# Autodesk Inventor assembly: ASY GBK 1310 long wall shield 4
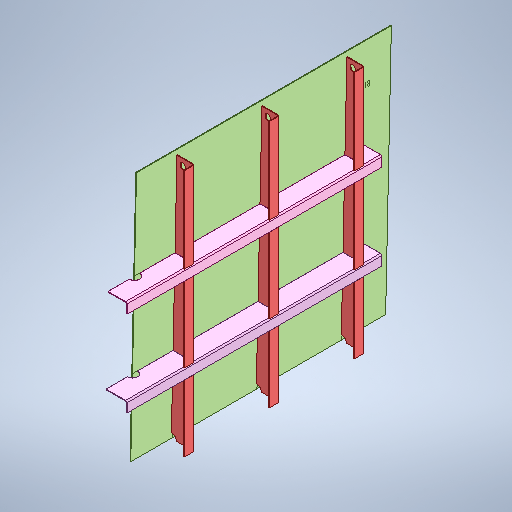
[picture p0: Inventor's stored thumbnail of the model, 512x512]
Saved by Autodesk Inventor 2026 (Build 300175000, 175)
## iProperties
Created: 2026-05-07
Part Number: ASY GBK 1310 long wall shield 4
Document SubType Name: Assembly
Designer: pokla
Mass: 107756 g
Surface Area: 69611.7 cm^2
Volume: 13726.9 cm^3
Stock Number: 1311
Author: admin
## Documents named in this file (6)
- C:\Users\pokla\Documents\Inventor\GBK-Gubkinskiy\ASY GBK 1310 long wall shield 4.iam
- C:\Users\pokla\Documents\Inventor\GBK-Gubkinskiy\07.1 GBK shield.ipt
- C:\Users\pokla\Documents\Inventor\GBK-Gubkinskiy\GBK 0301 third rib.ipt
- C:\Users\pokla\Documents\Inventor\GBK-Gubkinskiy\GBK 0302 stringer 7.ipt
- C:\Users\pokla\Documents\Inventor\GBK-Gubkinskiy\GBK 0303 stringer 8.ipt
- C:\Users\pokla\Documents\Inventor\GBK-Gubkinskiy\GBK 0101 main rib.ipt
## Components (6 placed, 4 different names)
1. GBK 0302 stringer 7.ipt:1
2. GBK 0303 stringer 8.ipt:1 — Заподлицо:1
3. 07.1 GBK shield.ipt:1 — Заподлицо:1, Совмещение:3
4. GBK 0301 third rib.ipt:1 — Совмещение:4, Заподлицо:2
5. GBK 0301 third rib.ipt:2
6. GBK 0301 third rib.ipt:3
## Component patterns: (3 elements, first: GBK 0301 third rib.ipt:1)
## Relationships (8: Mate 4, WeldJoint 2, Flush 2)
- [Mate]: 07.1 GBK shield.ipt:1 ↔ GBK 0301 third rib.ipt:1
- [Mate]: 07.1 GBK shield.ipt:1 ↔ GBK 0301 third rib.ipt:1
- [WeldJoint] (4 mm): GBK 0302 stringer 7.ipt:1 ↔ GBK 0301 third rib.ipt:1
- [WeldJoint] (4 mm): GBK 0303 stringer 8.ipt:1 ↔ GBK 0301 third rib.ipt:1
- Заподлицо:1 [Flush] (155 mm): GBK 0303 stringer 8.ipt:1 ↔ 07.1 GBK shield.ipt:1
- Совмещение:3 [Mate]: 07.1 GBK shield.ipt:1
- Совмещение:4 [Mate]: GBK 0301 third rib.ipt:1
- Заподлицо:2 [Flush]: GBK 0301 third rib.ipt:1
## Named parameters: Шаг_шпангоутов = 496.66667 mm
